# Autodesk Inventor assembly: sumobotLIDAR
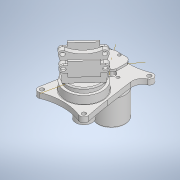
[picture p0: Inventor's stored thumbnail of the model, 180x180]
Saved by Autodesk Inventor 2022 (Build 260153070, 153G)
## iProperties
Created: 2021-10-27
Part Number: sumobotLIDAR
Document SubType Name: Assembly
Designer: a laptop
Mass: 24.9045 g
Surface Area: 154.1 cm^2
Volume: 24.9045 cm^3
Density: 1 g/cm^3
Author: a laptop
## Documents named in this file (9)
- C:\Users\a laptop\Desktop\sumobotLIDAR\sumobotLIDAR.iam
- C:\Users\a laptop\Desktop\sumobotLIDAR\MOTOR.ipt
- C:\Users\a laptop\Desktop\sumobotLIDAR\SRM-12-06A.ipt
- C:\Users\a laptop\Desktop\sumobotLIDAR\Adapterlowerplate.ipt
- C:\Users\a laptop\Desktop\sumobotLIDAR\608ZZ bearing.ipt
- C:\Users\a laptop\Desktop\sumobotLIDAR\Adapterupperplate.ipt
- C:\Users\a laptop\Desktop\sumobotLIDAR\VL53L1X board.ipt
- C:\Users\a laptop\Desktop\sumobotLIDAR\VL53L1X board_MIR1.ipt
- C:\Users\a laptop\Desktop\sumobotLIDAR\AS5600.ipt
## Components (8 placed, 8 different names)
1. MOTOR:1 — Angle:1, Flush:1, Mate:5, Mate:6, Mate:7, Tangent:1, Flush:3, Mate:18, Mate:32
2. SRM-12-06A:1 — Angle:1, Flush:1, Mate:1, Mate:2, Mate:10, Mate:13, Tangent:1, Mate:14, Mate:17
3. Adapterlowerplate:1 — Flush:3, Mate:16, Mate:17, Mate:18
4. 608ZZ bearing:1 — Mate:15, Mate:16, Flush:4, Rotational:1
5. Adapterupperplate:1 — Flush:4, Rotational:1, Mate:19, Mate:20, Mate:21, Flush:5, Mate:22, Mate:23, Flush:6
6. VL53L1X board:1 — Mate:19, Mate:20, Flush:5
7. VL53L1X board_MIR1:1 — Mate:22, Mate:23, Mate:24
8. AS5600:1 — Mate:25, Mate:26, Mate:27, Mate:28, Angle:4
## Relationships (44: Mate 32, Flush 6, Angle 4, Tangent 1, RevoluteJoint 1)
- Angle:1 (180 deg): MOTOR:1 ↔ SRM-12-06A:1
- Flush:1: MOTOR:1 ↔ SRM-12-06A:1
- Mate:1: SRM-12-06A:1
- Mate:2: SRM-12-06A:1
- Mate:3
- Mate:4
- Mate:5: MOTOR:1
- Mate:6: MOTOR:1
- Mate:7: MOTOR:1
- Mate:8
- Mate:9
- Flush:2 (17 mm)
- Angle:2 (180 deg)
- Mate:10: SRM-12-06A:1
- Mate:11
- Mate:12
- Angle:3 (90 deg)
- Mate:13: SRM-12-06A:1
- Tangent:1: MOTOR:1 ↔ SRM-12-06A:1
- Flush:3: MOTOR:1 ↔ Adapterlowerplate:1
- Mate:14: SRM-12-06A:1
- Mate:15: 608ZZ bearing:1
- Mate:16: Adapterlowerplate:1 ↔ 608ZZ bearing:1
- Flush:4: 608ZZ bearing:1 ↔ Adapterupperplate:1
- Rotational:1 [RevoluteJoint]: 608ZZ bearing:1 ↔ Adapterupperplate:1
- Mate:17: SRM-12-06A:1 ↔ Adapterlowerplate:1
- Mate:18: MOTOR:1 ↔ Adapterlowerplate:1
- Mate:19 (5 mm): Adapterupperplate:1 ↔ VL53L1X board:1
- Mate:20 (8 mm): Adapterupperplate:1 ↔ VL53L1X board:1
- Mate:21: Adapterupperplate:1
- Flush:5: Adapterupperplate:1 ↔ VL53L1X board:1
- Mate:22: Adapterupperplate:1 ↔ VL53L1X board_MIR1:1
- Mate:23: Adapterupperplate:1 ↔ VL53L1X board_MIR1:1
- Flush:6: Adapterupperplate:1
- Mate:24: VL53L1X board_MIR1:1
- Mate:25: AS5600:1
- Mate:26: AS5600:1
- Mate:27: AS5600:1
- Mate:28: AS5600:1
- Mate:29
- Mate:30
- Mate:31
- Angle:4 (0 deg): AS5600:1
- Mate:32: MOTOR:1
